# Autodesk Inventor assembly: Conjunto TapaVaso con Vaso
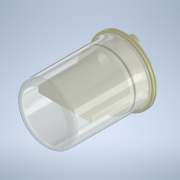
[picture p0: Inventor's stored thumbnail of the model, 180x180]
Saved by Autodesk Inventor 2020.3 (Build 243373000, 373)
## iProperties
Created: 2020-06-22
Part Number: Conjunto TapaVaso con Vaso
Document SubType Name: Assembly
Designer: Bruno
Author: Bruno
## Documents named in this file (12)
- C:\Users\Bruno\Desktop\CNAF\CNAF-3\Conjunto TapaVaso con Vaso.iam
- C:\Users\Bruno\Desktop\CNAF\CNAF-3\Cuerpo Tapa Sin Paleta.ipt
- C:\Users\Bruno\Desktop\CNAF\CNAF-3\Paleta.ipt
- C:\Users\Bruno\Desktop\CNAF\CNAF-3\Oring 2-019.ipt
- C:\Users\Bruno\Desktop\CNAF\CNAF-3\Oring 2-026.ipt
- C:\Users\Bruno\Desktop\CNAF\CNAF-3\Conector Tapa-Corrugado V2.ipt
- C:\Users\Bruno\Desktop\CNAF\CNAF-3\Conector Tapa-Tubo calefaccionado V2 (M33).ipt
- C:\Users\Bruno\Desktop\CNAF\CNAF-3\Oring 2-018 Deform.ipt
- C:\Users\Bruno\Desktop\CNAF\CNAF-3\Oring 2-022.ipt
- C:\Users\Bruno\Desktop\CNAF\CNAF-3\Perno Parker DIN912 M4x0.7x16-8.8.ipt
- C:\Users\Bruno\Desktop\CNAF\CNAF-3\Oring 2-151 Deform.ipt
- C:\Users\Bruno\Desktop\CNAF\CNAF-3\Vaso precipitado 600ml-De90-Di84-H120.ipt
## Components (11 placed, 11 different names)
1. Cuerpo Tapa Sin Paleta:1 — Cylindrical:3, Cylindrical:8, Cylindrical:9, Cylindrical:10, Cylindrical:11, Cylindrical:14, Cylindrical:15, Cylindrical:16
2. Paleta:1 — Cylindrical:3
3. Oring 2-019:1 — Cylindrical:8
4. Oring 2-026:1 — Cylindrical:9
5. Conector Tapa-Corrugado V2:1 — Cylindrical:10, Cylindrical:12
6. Conector Tapa-Tubo calefaccionado V2 (M33):1 — Cylindrical:11, Cylindrical:13
7. Oring 2-018 Deform:1 — Cylindrical:12
8. Oring 2-022:1 — Cylindrical:13
9. Perno Parker DIN912 M4x0.7x16-8.8:1 — Cylindrical:14
10. Oring 2-151 Deform:1 — Cylindrical:15
11. Vaso precipitado 600ml-De90-Di84-H120:1 — Cylindrical:16
## Relationships (10: CylindricalJoint 10)
- Cylindrical:3: Cuerpo Tapa Sin Paleta:1 ↔ Paleta:1
- Cylindrical:8: Cuerpo Tapa Sin Paleta:1 ↔ Oring 2-019:1
- Cylindrical:9: Cuerpo Tapa Sin Paleta:1 ↔ Oring 2-026:1
- Cylindrical:10: Cuerpo Tapa Sin Paleta:1 ↔ Conector Tapa-Corrugado V2:1
- Cylindrical:11: Cuerpo Tapa Sin Paleta:1 ↔ Conector Tapa-Tubo calefaccionado V2 (M33):1
- Cylindrical:12: Conector Tapa-Corrugado V2:1 ↔ Oring 2-018 Deform:1
- Cylindrical:13: Conector Tapa-Tubo calefaccionado V2 (M33):1 ↔ Oring 2-022:1
- Cylindrical:14: Cuerpo Tapa Sin Paleta:1 ↔ Perno Parker DIN912 M4x0.7x16-8.8:1
- Cylindrical:15: Cuerpo Tapa Sin Paleta:1 ↔ Oring 2-151 Deform:1
- Cylindrical:16: Cuerpo Tapa Sin Paleta:1 ↔ Vaso precipitado 600ml-De90-Di84-H120:1
